# Autodesk Inventor assembly: håndfang
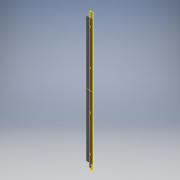
[picture p0: Inventor's stored thumbnail of the model, 180x180]
Saved by Autodesk Inventor 2018 (Build 220112000, 112)
## iProperties
Created: 2019-09-28
Part Number: håndfang
Document SubType Name: Assembly
Designer: loppen
Mass: 2419.67 g
Surface Area: 1505.05 cm^2
Volume: 308.239 cm^3
Density: 7.85 g/cm^3
Author: loppen
## Documents named in this file (4)
- Z:\trappe\håndfang\håndfang.iam
- Z:\trappe\håndfang\håndfang.ipt
- Z:\trappe\håndfang\afstandsstykke.ipt
- Z:\trappe\håndfang\afstandsstykke kort.ipt
## Components (7 placed, 3 different names)
1. håndfang:1 — Flush:1, Flush:2, Mate:1, Symmetry:1
2. håndfang:2 — Flush:1, Flush:2, Mate:1, Symmetry:1, Flush:3, Mate:2, Mate:3, Flush:4, Flush:5, Flush:6, Flush:7, Flush:8, Mate:4, Mate:5, Mate:6, Mate:7, Flush:9
3. afstandsstykke:1 — Mate:2, Mate:3, Flush:4, Mate:8
4. afstandsstykke kort:1 — Flush:8, Mate:7, Flush:9, Mate:9
5. afstandsstykke kort:2 — Flush:7, Mate:6, Mate:9
6. afstandsstykke kort:3 — Flush:6, Mate:5, Mate:10
7. afstandsstykke kort:4 — Flush:5, Mate:4, Mate:8, Mate:10
## Relationships (20: Mate 10, Flush 9, Symmetry 1)
- Flush:1: håndfang:1 ↔ håndfang:2
- Flush:2: håndfang:1 ↔ håndfang:2
- Mate:1 (-60 mm): håndfang:1 ↔ håndfang:2
- Symmetry:1: håndfang:1 ↔ håndfang:2
- Flush:3: håndfang:2
- Mate:2: håndfang:2 ↔ afstandsstykke:1
- Mate:3 (-40 mm): håndfang:2 ↔ afstandsstykke:1
- Flush:4: håndfang:2 ↔ afstandsstykke:1
- Flush:5: håndfang:2 ↔ afstandsstykke kort:4
- Flush:6: håndfang:2 ↔ afstandsstykke kort:3
- Flush:7: håndfang:2 ↔ afstandsstykke kort:2
- Flush:8: håndfang:2 ↔ afstandsstykke kort:1
- Mate:4: håndfang:2 ↔ afstandsstykke kort:4
- Mate:5: håndfang:2 ↔ afstandsstykke kort:3
- Mate:6: håndfang:2 ↔ afstandsstykke kort:2
- Mate:7: håndfang:2 ↔ afstandsstykke kort:1
- Mate:8 (20 mm): afstandsstykke:1 ↔ afstandsstykke kort:4
- Flush:9 (-60 mm): håndfang:2 ↔ afstandsstykke kort:1
- Mate:9 (326.317 mm): afstandsstykke kort:1 ↔ afstandsstykke kort:2
- Mate:10 (326.317 mm): afstandsstykke kort:3 ↔ afstandsstykke kort:4
